# Autodesk Inventor assembly: Vex Traction Wheel 6x1.5
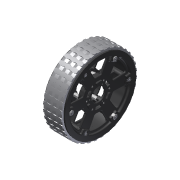
[picture p0: Inventor's stored thumbnail of the model, 180x180]
Saved by Autodesk Inventor 2013 (Build 170138000, 138)
## iProperties
Created: 2012-12-09
Part Number: Vex Traction Wheel 6x1.5
Document SubType Name: Assembly
Designer: Nemo
Author: Nemo
## Documents named in this file (7)
- H:\Nemo\Documents\Robotics\COTS Parts\Wheels\VexPro Traction Wheels\Vex Traction Wheel 6x1.5.iam
- H:\Nemo\Documents\Robotics\COTS Parts\Wheels\VexPro Traction Wheels\Components\Traction Wheel Body 6in.ipt
- H:\Nemo\Documents\Robotics\COTS Parts\Fasteners\8-32 locknut.ipt
- H:\Nemo\Documents\Robotics\COTS Parts\Fasteners\Hex Standoff 8-32 x1250.ipt
- H:\Nemo\Documents\Robotics\COTS Parts\Fasteners\8-32 BHCS x1750.ipt
- H:\Nemo\Documents\Robotics\COTS Parts\Wheels\VexPro Traction Wheels\Components\Traction Wheel extension 6in.ipt
- H:\Nemo\Documents\Robotics\COTS Parts\Wheels\VexPro Traction Wheels\Components\6 in Traction Tire.iam
## Components (24 placed, 6 different names)
1. Traction Wheel Body 6in:1 — Mate:1, Mate:2, Angle:1, Insert:1, Insert:2, Angle:2, Insert:3, Mate:6, Mate:7
2. Traction Wheel Body 6in:2 — Mate:3, Mate:4, Insert:4, Angle:3, Insert:5, Mate:8, Mate:12
3. Traction Wheel extension 6in:1 — Mate:5, Mate:6, Mate:7, Mate:8, Mate:9
4. 6 in Traction Tire:1 [sub-assembly] — Mate:10, Mate:11, Mate:12, Mate:18
5. 6 in Traction Tire:2 [sub-assembly] — Mate:13, Mate:14, Mate:17
6. 6 in Traction Tire:3 [sub-assembly] — Mate:15, Mate:16, Mate:17, Mate:18
7. Hex Standoff 8-32 x1250:1 — Angle:1, Insert:1
8. Hex Standoff 8-32 x1250:2
9. Hex Standoff 8-32 x1250:3
10. Hex Standoff 8-32 x1250:4
11. Hex Standoff 8-32 x1250:5
12. Hex Standoff 8-32 x1250:6
13. 8-32 BHCS x1750:1 — Insert:4
14. 8-32 locknut:2 — Angle:3, Insert:5
15. 8-32 BHCS x1750:4 — Insert:3
16. 8-32 locknut:1 — Insert:2, Angle:2
17. 8-32 BHCS x1750:2
18. 8-32 locknut:3
19. 8-32 BHCS x1750:5
20. 8-32 locknut:4
21. 8-32 BHCS x1750:3
22. 8-32 locknut:5
23. 8-32 BHCS x1750:6
24. 8-32 locknut:6
## Component patterns: (6 elements, first: Hex Standoff 8-32 x1250:1), (3 elements, first: 8-32 BHCS x1750:1 + 8-32 locknut:2 + 8-32 BHCS x1750:4 + 8-32 locknut:1)
## Relationships (26: Mate 18, Insert 5, Angle 3)
- Mate:1: Traction Wheel Body 6in:1
- Mate:2: Traction Wheel Body 6in:1
- Angle:1 (0 deg): Traction Wheel Body 6in:1 ↔ Hex Standoff 8-32 x1250:1
- Insert:1: Traction Wheel Body 6in:1 ↔ Hex Standoff 8-32 x1250:1
- Insert:2: Traction Wheel Body 6in:1 ↔ 8-32 locknut:1
- Angle:2 (0 deg): Traction Wheel Body 6in:1 ↔ 8-32 locknut:1
- Insert:3: Traction Wheel Body 6in:1 ↔ 8-32 BHCS x1750:4
- Mate:3: Traction Wheel Body 6in:2
- Mate:4: Traction Wheel Body 6in:2
- Insert:4: Traction Wheel Body 6in:2 ↔ 8-32 BHCS x1750:1
- Angle:3 (0 deg): Traction Wheel Body 6in:2 ↔ 8-32 locknut:2
- Insert:5: Traction Wheel Body 6in:2 ↔ 8-32 locknut:2
- Mate:5: Traction Wheel extension 6in:1
- Mate:6: Traction Wheel Body 6in:1 ↔ Traction Wheel extension 6in:1
- Mate:7: Traction Wheel Body 6in:1 ↔ Traction Wheel extension 6in:1
- Mate:8: Traction Wheel Body 6in:2 ↔ Traction Wheel extension 6in:1
- Mate:9: Traction Wheel extension 6in:1
- Mate:10: 6 in Traction Tire:1
- Mate:11: 6 in Traction Tire:1
- Mate:12: Traction Wheel Body 6in:2 ↔ 6 in Traction Tire:1
- Mate:13: 6 in Traction Tire:2
- Mate:14: 6 in Traction Tire:2
- Mate:15: 6 in Traction Tire:3
- Mate:16: 6 in Traction Tire:3
- Mate:17: 6 in Traction Tire:2 ↔ 6 in Traction Tire:3
- Mate:18: 6 in Traction Tire:1 ↔ 6 in Traction Tire:3
